# Autodesk Inventor assembly: longlongerarms
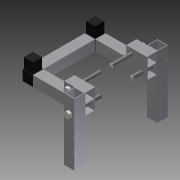
[picture p0: Inventor's stored thumbnail of the model, 180x180]
Saved by Autodesk Inventor 2011 (Build 150239000, 239)
## iProperties
Created: 2013-01-19
Part Number: longlongerarms
Document SubType Name: Assembly
Designer: Danny
Author: Danny
## Documents named in this file (6)
- C:\Users\Danny\Documents\GitHub\2013CAD\2013 robot\Spiderbot\longlongerarms.iam
- C:\Users\Danny\Documents\GitHub\2013CAD\2013 robot\Spiderbot\5 in 1-16.ipt
- C:\Users\Danny\Documents\GitHub\2013CAD\COTS parts\Plastic_Tubing_Connectors\3-way corner.ipt
- C:\Users\Danny\Documents\GitHub\2013CAD\2013 robot\Spiderbot\2 in 1-16.ipt
- C:\Users\Danny\Documents\GitHub\2013CAD\2013 robot\Spiderbot\6 in 1-16.ipt
- C:\Users\Danny\Documents\GitHub\2013CAD\2013 robot\Spiderbot\short hex bolt.ipt
## Components (13 placed, 5 different names)
1. 5 in 1-16:1 — Mate:1, Flush:1, Flush:2, Mate:2, Flush:3, Flush:4
2. 5 in 1-16:2 — Mate:3, Flush:5, Flush:6, Flush:9, Flush:10, Mate:5, Mate:8, Mate:11
3. 5 in 1-16:3 — Mate:4, Flush:7, Flush:8, Flush:11, Flush:12, Mate:6, Mate:10
4. 3-way corner:2 — Mate:2, Flush:3, Flush:4, Mate:4, Flush:7, Flush:8
5. 3-way corner:3 — Mate:1, Flush:1, Flush:2, Mate:3, Flush:5, Flush:6
6. 2 in 1-16:1 — Flush:11, Flush:12, Mate:6, Mate:9, Mate:13, Mate:16
7. 2 in 1-16:2 — Flush:9, Flush:10, Mate:5, Mate:7, Mate:18
8. 6 in 1-16:1 — Mate:11, Mate:12, Mate:17
9. 6 in 1-16:2 — Mate:13, Mate:14, Mate:15
10. Chassis_HexBolt_375x16x7_AndyMark_am-1055:1 — Mate:7, Mate:18
11. Chassis_HexBolt_375x16x7_AndyMark_am-1055:2 — Mate:8, Mate:12, Mate:17
12. Chassis_HexBolt_375x16x7_AndyMark_am-1055:3 — Mate:9, Mate:16
13. Chassis_HexBolt_375x16x7_AndyMark_am-1055:4 — Mate:10, Mate:14, Mate:15
## Relationships (30: Mate 18, Flush 12)
- Mate:1: 5 in 1-16:1 ↔ 3-way corner:3
- Flush:1: 5 in 1-16:1 ↔ 3-way corner:3
- Flush:2: 5 in 1-16:1 ↔ 3-way corner:3
- Mate:2: 5 in 1-16:1 ↔ 3-way corner:2
- Flush:3: 5 in 1-16:1 ↔ 3-way corner:2
- Flush:4: 5 in 1-16:1 ↔ 3-way corner:2
- Mate:3: 5 in 1-16:2 ↔ 3-way corner:3
- Flush:5: 5 in 1-16:2 ↔ 3-way corner:3
- Flush:6: 5 in 1-16:2 ↔ 3-way corner:3
- Mate:4: 5 in 1-16:3 ↔ 3-way corner:2
- Flush:7: 5 in 1-16:3 ↔ 3-way corner:2
- Flush:8: 5 in 1-16:3 ↔ 3-way corner:2
- Flush:9: 5 in 1-16:2 ↔ 2 in 1-16:2
- Flush:10: 5 in 1-16:2 ↔ 2 in 1-16:2
- Mate:5: 5 in 1-16:2 ↔ 2 in 1-16:2
- Flush:11: 5 in 1-16:3 ↔ 2 in 1-16:1
- Flush:12: 5 in 1-16:3 ↔ 2 in 1-16:1
- Mate:6: 5 in 1-16:3 ↔ 2 in 1-16:1
- Mate:7: 2 in 1-16:2 ↔ Chassis_HexBolt_375x16x7_AndyMark_am-1055:1
- Mate:8: 5 in 1-16:2 ↔ Chassis_HexBolt_375x16x7_AndyMark_am-1055:2
- Mate:9: 2 in 1-16:1 ↔ Chassis_HexBolt_375x16x7_AndyMark_am-1055:3
- Mate:10: 5 in 1-16:3 ↔ Chassis_HexBolt_375x16x7_AndyMark_am-1055:4
- Mate:11: 5 in 1-16:2 ↔ 6 in 1-16:1
- Mate:12: 6 in 1-16:1 ↔ Chassis_HexBolt_375x16x7_AndyMark_am-1055:2
- Mate:13: 2 in 1-16:1 ↔ 6 in 1-16:2
- Mate:14: 6 in 1-16:2 ↔ Chassis_HexBolt_375x16x7_AndyMark_am-1055:4
- Mate:15: 6 in 1-16:2 ↔ Chassis_HexBolt_375x16x7_AndyMark_am-1055:4
- Mate:16: 2 in 1-16:1 ↔ Chassis_HexBolt_375x16x7_AndyMark_am-1055:3
- Mate:17: 6 in 1-16:1 ↔ Chassis_HexBolt_375x16x7_AndyMark_am-1055:2
- Mate:18: 2 in 1-16:2 ↔ Chassis_HexBolt_375x16x7_AndyMark_am-1055:1
